# Autodesk Inventor assembly: Assembly_Cube_Z_Focus_MGN_manual_v3
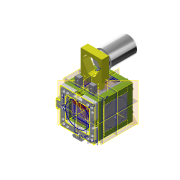
[picture p0: Inventor's stored thumbnail of the model, 180x180]
Saved by Autodesk Inventor 2022 (Build 260153000, 153)
## iProperties
Created: 2021-04-25
Part Number: Assembly_Cube_Z_Focus_MGN_manual_v3
Document SubType Name: Assembly
Designer: diederichbenedict
Author: diederichbenedict
## Documents named in this file (10)
- C:\Users\PrakashLab\Documents\UC2-INVENTOR-Git\uc2_v3\Assembly_Cube_Z_Focus_MGN_manual_v3.iam
- C:\Users\PrakashLab\Documents\UC2-Zstage\INVENTOR\Assembly_Cube_empty_IM_v3.iam
- C:\Users\PrakashLab\Documents\UC2-Zstage\INVENTOR\00_MGN12H, LINEAR GUIDE BLOCK.ipt
- C:\Users\PrakashLab\Documents\UC2-INVENTOR-Git\uc2_v3\00_Microscope_Objective_Lens10x.ipt
- C:\Users\PrakashLab\Documents\UC2-INVENTOR-Git\uc2_v3\30_Cube_Z_Focus_MGN_NEMA_adapter.ipt
- C:\Users\PrakashLab\Documents\UC2-INVENTOR-Git\uc2_v3\10_Base_puzzle_v3.ipt
- C:\Users\PrakashLab\Documents\UC2-Zstage\INVENTOR\30_Cube_Z_Focus_MGN_NEMA_rail.ipt
- C:\Users\PrakashLab\Documents\UC2-INVENTOR-Git\uc2_v3\30_Cube_Z_Focus_MGN12_manual_slide.ipt
- C:\Users\PrakashLab\Documents\UC2-INVENTOR-Git\uc2_v3\30_Cube_Z_Focus_MGN12_manual_gear_v3.ipt
- C:\Users\PrakashLab\Documents\UC2-INVENTOR-Git\uc2_v3\30_Cube_Z_Focus_MGN_manual_base_v3.ipt
## Components (10 placed, 9 different names)
1. Assembly_Cube_empty_IM_v3:1 [sub-assembly] — Flush:2, Flush:3, Mate:8, Flush:4, Flush:5, Mate:9, Insert:6
2. 00_MGN12H, LINEAR GUIDE BLOCK:1 — Flush:6, Mate:15, Mate:16, Insert:8
3. 30_Cube_Z_Focus_MGN_manual_base_v3:1 — Flush:2, Flush:3, Mate:8, Insert:7, Angle:1, Angle:2
4. Assembly_Cube_empty_IM_v3:2 [sub-assembly] — Flush:4, Flush:5, Mate:9, Mate:10
5. 00_Microscope_Objective_Lens10x:1 — Mate:10, Flush:6
6. 10_Base_puzzle_v3:1 — Insert:6
7. 30_Cube_Z_Focus_MGN_NEMA_rail:1 — Insert:7, Angle:1, Mate:15, Mate:16
8. 30_Cube_Z_Focus_MGN_NEMA_adapter:1 — Mate:12, Mate:13
9. 30_Cube_Z_Focus_MGN12_manual_slide:1 — Mate:12, Mate:13, Mate:14, Rotation:1, Insert:8, Angle:2, Mate:17
10. 30_Cube_Z_Focus_MGN12_manual_gear_v3:1 — Mate:14, Rotation:1, Mate:17
## Relationships (20: Mate 9, Flush 5, Insert 3, Angle 2, RelateRotation 1)
- Flush:2: Assembly_Cube_empty_IM_v3:1 ↔ 30_Cube_Z_Focus_MGN_manual_base_v3:1
- Flush:3: Assembly_Cube_empty_IM_v3:1 ↔ 30_Cube_Z_Focus_MGN_manual_base_v3:1
- Mate:8: Assembly_Cube_empty_IM_v3:1 ↔ 30_Cube_Z_Focus_MGN_manual_base_v3:1
- Flush:4: Assembly_Cube_empty_IM_v3:1 ↔ Assembly_Cube_empty_IM_v3:2
- Flush:5: Assembly_Cube_empty_IM_v3:1 ↔ Assembly_Cube_empty_IM_v3:2
- Mate:9 (0.1 mm): Assembly_Cube_empty_IM_v3:1 ↔ Assembly_Cube_empty_IM_v3:2
- Mate:10: Assembly_Cube_empty_IM_v3:2 ↔ 00_Microscope_Objective_Lens10x:1
- Flush:6 (-30 mm): 00_MGN12H, LINEAR GUIDE BLOCK:1 ↔ 00_Microscope_Objective_Lens10x:1
- Insert:6: Assembly_Cube_empty_IM_v3:1 ↔ 10_Base_puzzle_v3:1
- Mate:12: 30_Cube_Z_Focus_MGN_NEMA_adapter:1 ↔ 30_Cube_Z_Focus_MGN12_manual_slide:1
- Mate:13 (0.1 mm): 30_Cube_Z_Focus_MGN_NEMA_adapter:1 ↔ 30_Cube_Z_Focus_MGN12_manual_slide:1
- Mate:14: 30_Cube_Z_Focus_MGN12_manual_slide:1 ↔ 30_Cube_Z_Focus_MGN12_manual_gear_v3:1
- Rotation:1 [RelateRotation] (1 ul): 30_Cube_Z_Focus_MGN12_manual_slide:1 ↔ 30_Cube_Z_Focus_MGN12_manual_gear_v3:1
- Insert:7: 30_Cube_Z_Focus_MGN_manual_base_v3:1 ↔ 30_Cube_Z_Focus_MGN_NEMA_rail:1
- Angle:1 (0 deg): 30_Cube_Z_Focus_MGN_manual_base_v3:1 ↔ 30_Cube_Z_Focus_MGN_NEMA_rail:1
- Mate:15: 00_MGN12H, LINEAR GUIDE BLOCK:1 ↔ 30_Cube_Z_Focus_MGN_NEMA_rail:1
- Mate:16: 00_MGN12H, LINEAR GUIDE BLOCK:1 ↔ 30_Cube_Z_Focus_MGN_NEMA_rail:1
- Insert:8: 00_MGN12H, LINEAR GUIDE BLOCK:1 ↔ 30_Cube_Z_Focus_MGN12_manual_slide:1
- Angle:2 (0 deg): 30_Cube_Z_Focus_MGN_manual_base_v3:1 ↔ 30_Cube_Z_Focus_MGN12_manual_slide:1
- Mate:17 (0.3 mm): 30_Cube_Z_Focus_MGN12_manual_slide:1 ↔ 30_Cube_Z_Focus_MGN12_manual_gear_v3:1
